# Autodesk Inventor assembly: アームマウント
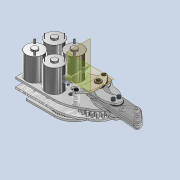
[picture p0: Inventor's stored thumbnail of the model, 180x180]
Saved by Autodesk Inventor 2020.4 (Build 244396000, 396)
## iProperties
Created: 2021-04-23
Part Number: アームマウント
Document SubType Name: Assembly
Designer: happy
Mass: 551.028 g
Surface Area: 834.365 cm^2
Volume: 164.292 cm^3
Density: 3.35396 g/cm^3
Author: happy
## Documents named in this file (39)
- C:\Users\happy\OneDrive\ドキュメント\賢一ファイル\SRDC\試作10-2\アセンブリ\アームマウント.iam
- C:\Users\happy\OneDrive\ドキュメント\賢一ファイル\SRDC\試作10-2\アームギア\外側フレーム.ipt
- C:\Users\happy\OneDrive\ドキュメント\賢一ファイル\SRDC\試作10-2\アームギア\最終段小ギア軸受け.ipt
- C:\Users\happy\OneDrive\ドキュメント\賢一ファイル\SRDC\試作10-2\アームギア\中間フレーム.ipt
- C:\Users\happy\OneDrive\ドキュメント\賢一ファイル\SRDC\試作10-2\モータ\アームモータマウント.ipt
- C:\Users\happy\OneDrive\ドキュメント\賢一ファイル\SRDC\試作10-2\モータ\アームモータマウント軸受けパーツ.ipt
- C:\Users\happy\OneDrive\ドキュメント\賢一ファイル\SRDC\試作10-2\モータ\RS-380.ipt
- C:\Users\happy\OneDrive\ドキュメント\賢一ファイル\SRDC\試作10-2\ねじ\m2.6 6mm キャップボルト.ipt
- C:\Users\happy\OneDrive\ドキュメント\賢一ファイル\SRDC\試作10-2\ねじ\m3皿ネジ6.ipt
- C:\Users\happy\OneDrive\ドキュメント\賢一ファイル\SRDC\試作10-2\スペーサ\12mm.ipt
- C:\Users\happy\OneDrive\ドキュメント\賢一ファイル\SRDC\試作10-2\スペーサ\5mm.ipt
- C:\Users\happy\OneDrive\ドキュメント\賢一ファイル\SRDC\試作10-2\軸受け\φ4φ8ベアリングa.ipt
- C:\Users\happy\OneDrive\ドキュメント\賢一ファイル\SRDC\試作10-2\ピン\φ4ピン　L20.ipt
- C:\Users\happy\OneDrive\ドキュメント\賢一ファイル\SRDC\試作10-2\ギア\ピニオン10.ipt
- C:\Users\happy\OneDrive\ドキュメント\賢一ファイル\SRDC\試作10-2\アームギア\1段目.iam
- C:\Users\happy\OneDrive\ドキュメント\賢一ファイル\SRDC\試作10-2\アームギア\2段目.iam
- C:\Users\happy\OneDrive\ドキュメント\賢一ファイル\SRDC\試作10-2\アームギア\3段目.iam
- C:\Users\happy\OneDrive\ドキュメント\賢一ファイル\SRDC\試作10-2\軸受け\ドライメッシュw6f12-14a.ipt
- C:\Users\happy\OneDrive\ドキュメント\賢一ファイル\SRDC\試作10-2\アームクランク\原動節2補助パーツ.ipt
- C:\Users\happy\OneDrive\ドキュメント\賢一ファイル\SRDC\試作10-2\アームクランク\従動節.ipt
- C:\Users\happy\OneDrive\ドキュメント\賢一ファイル\SRDC\試作10-2\アームクランク\揺動節.ipt
- C:\Users\happy\OneDrive\ドキュメント\賢一ファイル\SRDC\試作10-2\アームクランク\揺動節左.ipt
- C:\Users\happy\OneDrive\ドキュメント\賢一ファイル\SRDC\試作10-2\スペーサ\3mm.ipt
- C:\Users\happy\OneDrive\ドキュメント\賢一ファイル\SRDC\試作10-2\軸受け\オイレスw3f6-8n.ipt
- C:\Users\happy\OneDrive\ドキュメント\賢一ファイル\SRDC\試作10-2\軸受け\オイレスw10f8-10a.ipt
- C:\Users\happy\OneDrive\ドキュメント\賢一ファイル\SRDC\試作10-2\軸受け\オイレスw10f16-18a.ipt
- C:\Users\happy\OneDrive\ドキュメント\賢一ファイル\SRDC\試作10-2\アームクランク\原動節-従動節つなぎ.ipt
- C:\Users\happy\OneDrive\ドキュメント\賢一ファイル\SRDC\試作10-2\アームクランク\原動節外側.ipt
- C:\Users\happy\OneDrive\ドキュメント\賢一ファイル\SRDC\試作10-2\スペーサ\M4アルミスペーサ丸6.ipt
- C:\Users\happy\OneDrive\ドキュメント\賢一ファイル\SRDC\試作10-2\アームクランク\原動節固定部.ipt
- C:\Users\happy\OneDrive\ドキュメント\賢一ファイル\SRDC\試作10-2\軸受け\オイレスw5f8-10a.ipt
- C:\Users\happy\OneDrive\ドキュメント\賢一ファイル\SRDC\試作10-2\スペーサ\M4アルミスペーサー18.ipt
- C:\Users\happy\OneDrive\ドキュメント\賢一ファイル\SRDC\試作10-2\ねじ\M4ボタンボルト24.ipt
- C:\Users\happy\OneDrive\ドキュメント\賢一ファイル\SRDC\試作10-2\ねじ\M4ボタンボルト8.ipt
- C:\Users\happy\OneDrive\ドキュメント\賢一ファイル\SRDC\試作10-2\ねじ\M3キャップボルト 24.ipt
- C:\Users\happy\OneDrive\ドキュメント\賢一ファイル\SRDC\試作10-2\ねじ\M2-m3皿ネジ10 (1).ipt
- C:\Users\happy\OneDrive\ドキュメント\賢一ファイル\SRDC\試作10-2\ねじ\M3ボタンボルト6.ipt
- C:\Users\happy\OneDrive\ドキュメント\賢一ファイル\SRDC\試作10-2\アーム\アーム詰め物.ipt
- C:\Users\happy\OneDrive\ドキュメント\賢一ファイル\SRDC\試作10-2\スペーサ\16mm.ipt
## Components (75 placed, 38 different names)
1. 外側フレーム:1 — メイト:3, メイト:4, メイト:6, 挿入:30, 挿入:31, フラッシュ:1, フラッシュ:2, 挿入:83
2. 最終段小ギア軸受け:1 — 挿入:3, 挿入:4, 挿入:33
3. 中間フレーム:1 — メイト:1, メイト:2, メイト:3, メイト:4, メイト:5, メイト:6, 挿入:28, 挿入:29, 挿入:81, 挿入:82, 挿入:84
4. アームモータマウント:1 — 挿入:1, 挿入:2, 挿入:3, 挿入:4, メイト:1, メイト:2, メイト:5, 挿入:5, 挿入:6, 挿入:7, 挿入:8, 挿入:9, 挿入:10, 挿入:11, 挿入:12, 挿入:13, 挿入:14, 挿入:15, 挿入:16, 挿入:17, 挿入:18, 挿入:19, 挿入:20, 挿入:21, 挿入:22, 挿入:23, 挿入:24, 挿入:25, 挿入:26, 挿入:27, メイト:9, メイト:10, 挿入:44, 挿入:45, 挿入:46, 挿入:69, 挿入:71, 挿入:80, 挿入:85
5. アームモータマウント軸受けパーツ:1 — 挿入:1, 挿入:2, 挿入:32
6. RS-380:1 — 挿入:5, 挿入:6, 挿入:37
7. RS-380:2 — 挿入:11, 挿入:12, 挿入:34
8. RS-380:3 — 挿入:7, 挿入:8, 挿入:35
9. RS-380:4 — 挿入:9, 挿入:10, 挿入:36
10. m2.6 6mm キャップボルト:1 — 挿入:13
11. m2.6 6mm キャップボルト:2 — 挿入:14
12. m2.6 6mm キャップボルト:3 — 挿入:15
13. m2.6 6mm キャップボルト:4 — 挿入:16
14. m2.6 6mm キャップボルト:5 — 挿入:17
15. m2.6 6mm キャップボルト:6 — 挿入:18
16. m2.6 6mm キャップボルト:7 — 挿入:19
17. m2.6 6mm キャップボルト:8 — 挿入:20
18. m3皿ネジ6:1 — 挿入:21
19. m3皿ネジ6:2 — 挿入:22
20. m3皿ネジ6:3 — 挿入:23
21. m3皿ネジ6:4 — 挿入:25
22. m3皿ネジ6:5 — 挿入:26
23. m3皿ネジ6:6 — 挿入:27
24. m3皿ネジ6:7 — 挿入:24
25. 12mm:1 — 挿入:28
26. 5mm:1 — 挿入:29
27. φ4φ8ベアリングa:1 — 挿入:30, メイト:8, 挿入:41
28. φ4φ8ベアリングa:2 — 挿入:31, メイト:7
29. φ4φ8ベアリングa:3 — 挿入:32, 挿入:38
30. φ4φ8ベアリングa:4 — 挿入:33
31. φ4ピン　L20:1 — メイト:7, フラッシュ:1
32. φ4ピン　L20:2 — メイト:8, フラッシュ:2
33. ピニオン10:1 — 挿入:34
34. ピニオン10:2 — 挿入:35
35. ピニオン10:3 — 挿入:36
36. ピニオン10:4 — 挿入:37
37. 1段目:1 [sub-assembly] — 挿入:38
38. 2段目:1 [sub-assembly] — 挿入:41
39. 3段目:1 [sub-assembly] — メイト:9, メイト:10, 挿入:55, 挿入:57, 挿入:78, 挿入:79
40. ドライメッシュw6f12-14a:1 — 挿入:44
41. 原動節2補助パーツ:1 — 挿入:45
42. 従動節:1 — メイト:12, 挿入:50, 挿入:52
43. 揺動節:1 — メイト:12, 挿入:47, メイト:14, 挿入:56, 挿入:88, 挿入:89
44. 12mm:2 — 挿入:46
45. 揺動節左:1 — 挿入:48, メイト:14, 挿入:86, 挿入:87
46. 3mm:1 — 挿入:47, 挿入:48, 挿入:49
47. オイレスw3f6-8n:1 — 挿入:49, 挿入:50
48. オイレスw10f8-10a:1 — 挿入:52, メイト:15
49. オイレスw10f16-18a:1 — 挿入:55, 挿入:56, 挿入:58
50. 原動節-従動節つなぎ:1 — 挿入:57, 挿入:58, 挿入:59, 挿入:60
51. 原動節-従動節つなぎ:2 — 挿入:59, 挿入:60, 挿入:61, 挿入:62
52. 原動節外側:1 — 挿入:61, 挿入:62, 挿入:64, 挿入:76, 挿入:77
53. M4アルミスペーサ丸6:1 — 挿入:64, 挿入:67, 挿入:75
54. 原動節固定部:1 — 挿入:70, 挿入:72, 挿入:73, 挿入:74
55. オイレスw5f8-10a:1 — 挿入:67
56. M4アルミスペーサー18:2 — 挿入:69, 挿入:70
57. M4アルミスペーサー18:4 — 挿入:71, メイト:15, 挿入:72
58. M4ボタンボルト24:1 — 挿入:73
59. M4ボタンボルト24:2 — 挿入:74
60. M4ボタンボルト8:1 — 挿入:75
61. M3キャップボルト 24:1 — 挿入:76
62. M3キャップボルト 24:2 — 挿入:77
63. M2-m3皿ネジ10 (1):1 — 挿入:78
64. M2-m3皿ネジ10 (1):2 — 挿入:79
65. M3ボタンボルト6:1 — 挿入:80
66. M3ボタンボルト6:2 — 挿入:81
67. M3ボタンボルト6:3 — 挿入:82
68. M3ボタンボルト6:4 — 挿入:84
69. M3ボタンボルト6:6 — 挿入:83
70. M3ボタンボルト6:7 — 挿入:85
71. アーム詰め物:1 — 挿入:88, 挿入:89
72. アーム詰め物:2 — 挿入:86, 挿入:87, メイト:16, メイト:17, メイト:18, フラッシュ:3, フラッシュ:4, フラッシュ:5
73. 16mm:1 — メイト:16, フラッシュ:4
74. 16mm:2 — メイト:17, フラッシュ:5
75. 16mm:3 — メイト:18, フラッシュ:3
## Relationships (99: Insert 78, Mate 16, Flush 5)
- 挿入:1 [Insert]: アームモータマウント:1 ↔ アームモータマウント軸受けパーツ:1
- 挿入:2 [Insert]: アームモータマウント:1 ↔ アームモータマウント軸受けパーツ:1
- 挿入:3 [Insert]: 最終段小ギア軸受け:1 ↔ アームモータマウント:1
- 挿入:4 [Insert]: 最終段小ギア軸受け:1 ↔ アームモータマウント:1
- メイト:1 [Mate]: 中間フレーム:1 ↔ アームモータマウント:1
- メイト:2 [Mate]: 中間フレーム:1 ↔ アームモータマウント:1
- メイト:3 [Mate]: 外側フレーム:1 ↔ 中間フレーム:1
- メイト:4 [Mate]: 外側フレーム:1 ↔ 中間フレーム:1
- メイト:5 [Mate] (11 mm): 中間フレーム:1 ↔ アームモータマウント:1
- メイト:6 [Mate] (5 mm): 外側フレーム:1 ↔ 中間フレーム:1
- 挿入:5 [Insert]: アームモータマウント:1 ↔ RS-380:1
- 挿入:6 [Insert]: アームモータマウント:1 ↔ RS-380:1
- 挿入:7 [Insert]: アームモータマウント:1 ↔ RS-380:3
- 挿入:8 [Insert]: アームモータマウント:1 ↔ RS-380:3
- 挿入:9 [Insert]: アームモータマウント:1 ↔ RS-380:4
- 挿入:10 [Insert]: アームモータマウント:1 ↔ RS-380:4
- 挿入:11 [Insert]: アームモータマウント:1 ↔ RS-380:2
- 挿入:12 [Insert]: アームモータマウント:1 ↔ RS-380:2
- 挿入:13 [Insert]: アームモータマウント:1 ↔ m2.6 6mm キャップボルト:1
- 挿入:14 [Insert]: アームモータマウント:1 ↔ m2.6 6mm キャップボルト:2
- 挿入:15 [Insert]: アームモータマウント:1 ↔ m2.6 6mm キャップボルト:3
- 挿入:16 [Insert]: アームモータマウント:1 ↔ m2.6 6mm キャップボルト:4
- 挿入:17 [Insert]: アームモータマウント:1 ↔ m2.6 6mm キャップボルト:5
- 挿入:18 [Insert]: アームモータマウント:1 ↔ m2.6 6mm キャップボルト:6
- 挿入:19 [Insert]: アームモータマウント:1 ↔ m2.6 6mm キャップボルト:7
- 挿入:20 [Insert]: アームモータマウント:1 ↔ m2.6 6mm キャップボルト:8
- 挿入:21 [Insert]: アームモータマウント:1 ↔ m3皿ネジ6:1
- 挿入:22 [Insert]: アームモータマウント:1 ↔ m3皿ネジ6:2
- 挿入:23 [Insert]: アームモータマウント:1 ↔ m3皿ネジ6:3
- 挿入:24 [Insert]: アームモータマウント:1 ↔ m3皿ネジ6:7
- 挿入:25 [Insert]: アームモータマウント:1 ↔ m3皿ネジ6:4
- 挿入:26 [Insert]: アームモータマウント:1 ↔ m3皿ネジ6:5
- 挿入:27 [Insert]: アームモータマウント:1 ↔ m3皿ネジ6:6
- 挿入:28 [Insert]: 中間フレーム:1 ↔ 12mm:1
- 挿入:29 [Insert]: 中間フレーム:1 ↔ 5mm:1
- 挿入:30 [Insert]: 外側フレーム:1 ↔ φ4φ8ベアリングa:1
- 挿入:31 [Insert]: 外側フレーム:1 ↔ φ4φ8ベアリングa:2
- 挿入:32 [Insert]: アームモータマウント軸受けパーツ:1 ↔ φ4φ8ベアリングa:3
- 挿入:33 [Insert]: 最終段小ギア軸受け:1 ↔ φ4φ8ベアリングa:4
- メイト:7 [Mate]: φ4φ8ベアリングa:2 ↔ φ4ピン　L20:1
- メイト:8 [Mate]: φ4φ8ベアリングa:1 ↔ φ4ピン　L20:2
- 挿入:34 [Insert]: RS-380:2 ↔ ピニオン10:1
- 挿入:35 [Insert]: RS-380:3 ↔ ピニオン10:2
- 挿入:36 [Insert]: RS-380:4 ↔ ピニオン10:3
- 挿入:37 [Insert]: RS-380:1 ↔ ピニオン10:4
- 挿入:38 [Insert]: φ4φ8ベアリングa:3 ↔ 1段目:1
- 挿入:41 [Insert]: φ4φ8ベアリングa:1 ↔ 2段目:1
- フラッシュ:1 [Flush] (1 mm): 外側フレーム:1 ↔ φ4ピン　L20:1
- フラッシュ:2 [Flush] (1 mm): 外側フレーム:1 ↔ φ4ピン　L20:2
- メイト:9 [Mate] (1 mm): アームモータマウント:1 ↔ 3段目:1
- メイト:10 [Mate]: アームモータマウント:1 ↔ 3段目:1
- 挿入:44 [Insert]: アームモータマウント:1 ↔ ドライメッシュw6f12-14a:1
- 挿入:45 [Insert]: アームモータマウント:1 ↔ 原動節2補助パーツ:1
- メイト:12 [Mate]: 従動節:1 ↔ 揺動節:1
- 挿入:46 [Insert]: アームモータマウント:1 ↔ 12mm:2
- 挿入:47 [Insert]: 揺動節:1 ↔ 3mm:1
- 挿入:48 [Insert]: 揺動節左:1 ↔ 3mm:1
- 挿入:49 [Insert]: 3mm:1 ↔ オイレスw3f6-8n:1
- 挿入:50 [Insert]: 従動節:1 ↔ オイレスw3f6-8n:1
- メイト:14 [Mate]: 揺動節:1 ↔ 揺動節左:1
- 挿入:52 [Insert]: 従動節:1 ↔ オイレスw10f8-10a:1
- 挿入:55 [Insert]: 3段目:1 ↔ オイレスw10f16-18a:1
- 挿入:56 [Insert]: 揺動節:1 ↔ オイレスw10f16-18a:1
- 挿入:57 [Insert]: 3段目:1 ↔ 原動節-従動節つなぎ:1
- 挿入:58 [Insert]: オイレスw10f16-18a:1 ↔ 原動節-従動節つなぎ:1
- 挿入:59 [Insert]: 原動節-従動節つなぎ:1 ↔ 原動節-従動節つなぎ:2
- 挿入:60 [Insert]: 原動節-従動節つなぎ:1 ↔ 原動節-従動節つなぎ:2
- 挿入:61 [Insert]: 原動節-従動節つなぎ:2 ↔ 原動節外側:1
- 挿入:62 [Insert]: 原動節-従動節つなぎ:2 ↔ 原動節外側:1
- 挿入:64 [Insert]: 原動節外側:1 ↔ M4アルミスペーサ丸6:1
- 挿入:67 [Insert]: M4アルミスペーサ丸6:1 ↔ オイレスw5f8-10a:1
- 挿入:69 [Insert]: アームモータマウント:1 ↔ M4アルミスペーサー18:2
- 挿入:70 [Insert]: 原動節固定部:1 ↔ M4アルミスペーサー18:2
- 挿入:71 [Insert]: アームモータマウント:1 ↔ M4アルミスペーサー18:4
- メイト:15 [Mate]: オイレスw10f8-10a:1 ↔ M4アルミスペーサー18:4
- 挿入:72 [Insert]: 原動節固定部:1 ↔ M4アルミスペーサー18:4
- 挿入:73 [Insert]: 原動節固定部:1 ↔ M4ボタンボルト24:1
- 挿入:74 [Insert]: 原動節固定部:1 ↔ M4ボタンボルト24:2
- 挿入:75 [Insert]: M4アルミスペーサ丸6:1 ↔ M4ボタンボルト8:1
- 挿入:76 [Insert]: 原動節外側:1 ↔ M3キャップボルト 24:1
- 挿入:77 [Insert]: 原動節外側:1 ↔ M3キャップボルト 24:2
- 挿入:78 [Insert]: 3段目:1 ↔ M2-m3皿ネジ10 (1):1
- 挿入:79 [Insert]: 3段目:1 ↔ M2-m3皿ネジ10 (1):2
- 挿入:80 [Insert]: アームモータマウント:1 ↔ M3ボタンボルト6:1
- 挿入:81 [Insert]: 中間フレーム:1 ↔ M3ボタンボルト6:2
- 挿入:82 [Insert]: 中間フレーム:1 ↔ M3ボタンボルト6:3
- 挿入:83 [Insert]: 外側フレーム:1 ↔ M3ボタンボルト6:6
- 挿入:84 [Insert]: 中間フレーム:1 ↔ M3ボタンボルト6:4
- 挿入:85 [Insert]: アームモータマウント:1 ↔ M3ボタンボルト6:7
- 挿入:86 [Insert]: 揺動節左:1 ↔ アーム詰め物:2
- 挿入:87 [Insert]: 揺動節左:1 ↔ アーム詰め物:2
- 挿入:88 [Insert]: 揺動節:1 ↔ アーム詰め物:1
- 挿入:89 [Insert]: 揺動節:1 ↔ アーム詰め物:1
- メイト:16 [Mate]: アーム詰め物:2 ↔ 16mm:1
- メイト:17 [Mate]: アーム詰め物:2 ↔ 16mm:2
- メイト:18 [Mate]: アーム詰め物:2 ↔ 16mm:3
- フラッシュ:3 [Flush] (-1 mm): アーム詰め物:2 ↔ 16mm:3
- フラッシュ:4 [Flush] (-1 mm): アーム詰め物:2 ↔ 16mm:1
- フラッシュ:5 [Flush] (-1 mm): アーム詰め物:2 ↔ 16mm:2
